# Autodesk Inventor assembly: Carriage_Assembly
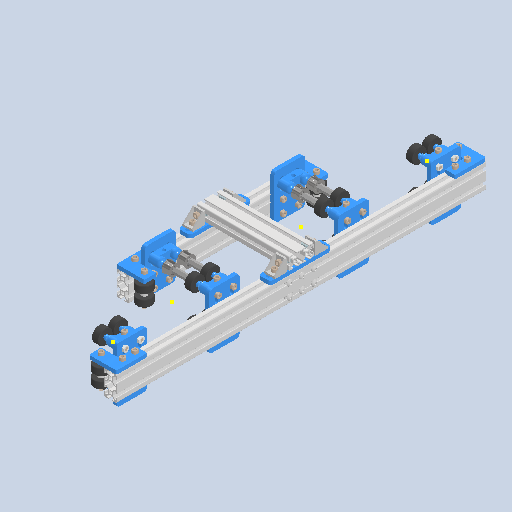
[picture p0: Inventor's stored thumbnail of the model, 512x512]
Saved by Autodesk Inventor 2022 (Build 260153000, 153)
## iProperties
Created: 2021-09-08
Part Number: Carriage_Assembly
Document SubType Name: Assembly
Designer: Jorian Brusind
Author: Jorian Brusind
## Documents named in this file (16)
- C:\Users\Jorian Brusind\Documents\GitHub\HyperRail\Inventor Files\Carriage_Assembly.iam
- C:\Users\Jorian Brusind\Documents\GitHub\HyperRail\Inventor Files\8020_Sets\IPT_20_Series\IPT_20_Series\20-2040_150mm.ipt
- C:\Users\Jorian Brusind\Documents\GitHub\HyperRail\Inventor Files\8020_Sets\IPT_20_Series\Extra_20_Series\8020_14056m\14056_m.ipt
- C:\Users\Jorian Brusind\Documents\GitHub\HyperRail\Inventor Files\Buffer.iam
- C:\Users\Jorian Brusind\Documents\GitHub\HyperRail\Inventor Files\Metric Spacer_Standoffs\hex spacer standoff nut M5 L30.ipt
- C:\Users\Jorian Brusind\Documents\GitHub\HyperRail\Inventor Files\Carriage_Horizontal_Spacer.ipt
- C:\Users\Jorian Brusind\Documents\GitHub\HyperRail\Inventor Files\8020_Sets\IPT_20_Series\IPT_20_Series\20-2040_400mm.ipt
- C:\Users\Jorian Brusind\Documents\GitHub\HyperRail\Inventor Files\Buffer_L.iam
- C:\Users\Jorian Brusind\Documents\GitHub\HyperRail\Inventor Files\Metric bolt\Bolt M5 10mm.ipt
- C:\Users\Jorian Brusind\Documents\GitHub\HyperRail\Inventor Files\din-508-t-slot-nut-t-nut-m4-m42-2.snapshot.3\STEPS\DIN 508, T-Slot Nut M5.ipt
- C:\Users\Jorian Brusind\Documents\GitHub\HyperRail\Inventor Files\8020_Sets\IPT_20_Series\IPT_20_Series\20-2040_300mm.ipt
- C:\Users\Jorian Brusind\Documents\GitHub\HyperRail\Inventor Files\5537T425_T-SLOTTED FRAMING.ipt
- C:\Users\Jorian Brusind\Documents\GitHub\HyperRail\Inventor Files\X_CarriageFWD_V2_1.iam
- C:\Users\Jorian Brusind\Documents\GitHub\HyperRail\Inventor Files\X_CarriageFWDBearing_V2_1_Short.iam
- C:\Users\Jorian Brusind\Documents\GitHub\HyperRail\Inventor Files\X_CarriageBWD_V2_0.iam
- C:\Users\Jorian Brusind\Documents\GitHub\HyperRail\Inventor Files\Metric bolt\Bolt M5 12mm.ipt
## Components (106 placed, 15 different names)
1. 20-2040_150mm:1 — Mate:20, Mate:21, Mate:22, Mate:23, Mate:80, Flush:33, Flush:94, Flush:96, Flush:99, Flush:102, Flush:114, Flush:124, Mate:311, Flush:186
2. 14056_m:1 — Mate:21, Flush:26, Flush:38, Mate:167, Mate:170, Mate:376, Mate:377
3. 14056_m:2 — Mate:20, Flush:26, Mate:70, Flush:37, Mate:164, Mate:165, Mate:379
4. 14056_m:3 — Mate:22, Flush:13, Mate:156, Mate:158, Flush:115, Mate:383
5. 14056_m:4 — Mate:23, Flush:13, Mate:72, Mate:159, Mate:161, Flush:114, Flush:115, Flush:116, Mate:381
6. Buffer:2 [sub-assembly] — Mate:86, Flush:55, Mate:202, Mate:203, Mate:206, Mate:207, Flush:120, Mate:293
7. Buffer:3 [sub-assembly] — Mate:196, Mate:197, Mate:198, Mate:199, Flush:127, Flush:128, Mate:310, Mate:368
8. Carriage_Horizontal_Spacer:1 — Mate:72, Mate:79, Mate:80, Flush:116, Flush:117
9. Carriage_Horizontal_Spacer:2 — Mate:70, Flush:37, Flush:38, Flush:117, Mate:290, Flush:123
10. 20-2040_400mm:1 — Mate:75, Mate:76, Mate:79, Flush:33, Mate:86, Flush:55, Mate:140, Flush:71, Flush:97, Flush:98, Flush:100, Flush:101, Flush:103, Flush:104, Flush:118, Flush:120, Mate:291, Mate:292, Flush:129, Flush:130, Mate:355, Mate:364, Flush:185, Flush:186
11. hex spacer standoff nut M5 L30:1 — Mate:295, Mate:305
12. hex spacer standoff nut M5 L30:2 — Mate:298, Mate:302
13. hex spacer standoff nut M5 L30:3 — Mate:296, Mate:306
14. hex spacer standoff nut M5 L30:4 — Mate:297, Mate:301
15. Buffer_L:1 [sub-assembly] — Mate:192, Mate:193, Mate:194, Mate:195, Flush:125, Flush:126, Mate:309, Mate:367
16. Buffer_L:2 [sub-assembly] — Mate:140, Flush:71, Mate:200, Mate:201, Mate:204, Mate:205, Flush:118, Mate:294
17. Bolt M5 10mm:1 — Mate:156, Mate:158, Mate:231
18. Bolt M5 10mm:3 — Mate:164, Mate:165, Mate:227
19. Bolt M5 10mm:6 — Mate:167, Mate:170, Mate:224
20. Bolt M5 10mm:8 — Mate:159, Mate:161, Mate:233
21. Bolt M5 10mm:9 — Mate:192, Mate:195, Mate:225
22. Bolt M5 10mm:10 — Mate:193, Mate:194, Mate:226
23. Bolt M5 10mm:11 — Mate:202, Mate:206, Mate:230
24. Bolt M5 10mm:12 — Mate:201, Mate:205, Mate:236
25. Bolt M5 10mm:13 — Mate:203, Mate:207, Mate:229
26. Bolt M5 10mm:14 — Mate:200, Mate:204, Mate:235
27. Bolt M5 10mm:15 — Mate:197, Mate:198, Mate:371
28. Bolt M5 10mm:16 — Mate:196, Mate:199, Mate:220
29. DIN 508, T-Slot Nut M5:1 — Mate:220, Mate:370
30. DIN 508, T-Slot Nut M5:2 — Mate:373, Mate:375
31. DIN 508, T-Slot Nut M5:4 — Mate:225
32. DIN 508, T-Slot Nut M5:5 — Mate:226, Mate:369
33. DIN 508, T-Slot Nut M5:6 — Mate:227, Flush:96
34. DIN 508, T-Slot Nut M5:7 — Mate:224, Flush:94
35. DIN 508, T-Slot Nut M5:8 — Mate:374, Mate:378
36. DIN 508, T-Slot Nut M5:10 — Mate:229, Flush:98
37. DIN 508, T-Slot Nut M5:11 — Mate:230, Flush:97
38. DIN 508, T-Slot Nut M5:12 — Flush:100, Mate:382
39. DIN 508, T-Slot Nut M5:13 — Mate:231, Flush:99
40. DIN 508, T-Slot Nut M5:14 — Mate:233, Flush:102
41. DIN 508, T-Slot Nut M5:15 — Flush:101, Mate:380
42. DIN 508, T-Slot Nut M5:16 — Mate:235, Flush:103
43. DIN 508, T-Slot Nut M5:17 — Mate:236, Flush:104
44. 20-2040_300mm:1 — Mate:283, Mate:284, Mate:285, Mate:286, Mate:287, Mate:288, Mate:289, Flush:121, Flush:122, Mate:290, Flush:123, Flush:124, Flush:127, Flush:128, Mate:299, Mate:308, Mate:311, Mate:318, Mate:319, Mate:368, Mate:370, Mate:372, Mate:373
45. 20-2040_300mm:2 — Mate:289, Flush:121, Flush:122, Flush:125, Flush:126, Mate:300, Mate:307, Mate:346, Flush:185, Mate:367, Mate:369, Mate:374, Mate:384, Mate:385
46. 5537T425_T-SLOTTED FRAMING:1 — Mate:283, Mate:284, Mate:285
47. 5537T425_T-SLOTTED FRAMING:2 — Mate:286, Mate:287, Mate:288
48. X_CarriageFWD_V2_1:1 [sub-assembly] — Mate:300, Mate:301, Mate:302, Flush:133, Mate:303, Flush:134, Flush:137, Flush:138, Flush:139, Flush:140, Mate:334, Mate:335, Mate:336, Mate:337, Mate:366, Flush:188, Flush:189, Flush:193
49. X_CarriageFWD_V2_1:2 [sub-assembly] — Mate:299, Mate:304, Mate:305, Mate:306, Flush:135, Flush:136, Flush:137, Flush:140, Flush:141, Flush:143, Mate:316, Mate:317, Mate:320, Mate:321, Flush:187, Flush:188, Flush:193
50. X_CarriageFWDBearing_V2_1_Short:1 [sub-assembly] — Mate:291, Flush:129, Mate:293, Mate:297, Mate:298, Flush:133, Mate:303, Flush:142, Mate:351, Mate:352, Mate:353, Mate:354
51. X_CarriageFWDBearing_V2_1_Short:2 [sub-assembly] — Mate:292, Flush:130, Mate:294, Mate:295, Mate:296, Mate:304, Flush:142, Flush:143, Mate:360, Mate:361, Mate:362, Mate:363, Mate:365
52. X_CarriageBWD_V2_0:1 [sub-assembly] — Mate:307, Flush:134, Mate:309, Flush:138, Flush:139, Mate:342, Mate:343, Mate:344, Mate:345, Flush:189
53. X_CarriageBWD_V2_0:2 [sub-assembly] — Mate:308, Flush:135, Mate:310, Flush:136, Flush:141, Mate:326, Mate:327, Mate:328, Mate:329, Flush:187
54. Bolt M5 10mm:17 — Mate:316, Flush:180
55. DIN 508, T-Slot Nut M5:18 — Mate:318
56. Bolt M5 10mm:18 — Mate:317, Flush:179, Flush:181
57. DIN 508, T-Slot Nut M5:19 — Mate:319
58. Bolt M5 10mm:19 — Mate:320, Flush:178
59. DIN 508, T-Slot Nut M5:20 — Flush:147, Flush:148, Flush:156
60. Bolt M5 10mm:20 — Mate:321, Flush:177, Flush:178, Flush:179, Flush:180
61. DIN 508, T-Slot Nut M5:21 — Flush:148
62. Bolt M5 10mm:21 — Mate:327, Flush:182
63. DIN 508, T-Slot Nut M5:22 — Flush:146
64. Bolt M5 10mm:22 — Mate:329, Flush:181, Flush:182, Flush:183, Flush:184
65. DIN 508, T-Slot Nut M5:23 — Flush:145, Flush:146
66. Bolt M5 10mm:23 — Mate:326, Flush:184
67. DIN 508, T-Slot Nut M5:24 — Flush:144, Flush:145
68. Bolt M5 10mm:24 — Mate:328, Flush:183
69. DIN 508, T-Slot Nut M5:25 — Flush:144, Flush:147
70. Bolt M5 10mm:25 — Mate:334, Flush:170, Mate:385
71. DIN 508, T-Slot Nut M5:26 — Flush:154, Flush:155
72. Bolt M5 10mm:26 — Mate:335, Flush:172
73. DIN 508, T-Slot Nut M5:27 — Flush:155, Flush:156
74. Bolt M5 10mm:27 — Mate:336, Mate:366, Flush:170, Flush:171, Flush:172, Flush:173, Mate:384
75. DIN 508, T-Slot Nut M5:28 — Flush:153, Flush:154
76. Bolt M5 10mm:28 — Mate:337, Flush:171, Flush:177
77. DIN 508, T-Slot Nut M5:29 — Flush:152, Flush:153
78. Bolt M5 10mm:29 — Mate:342, Flush:174
79. DIN 508, T-Slot Nut M5:30 — Flush:150, Flush:151, Flush:152
80. Bolt M5 10mm:30 — Mate:343, Flush:173, Flush:174, Flush:175, Flush:176
81. DIN 508, T-Slot Nut M5:31 — Flush:150
82. Bolt M5 10mm:31 — Mate:344, Flush:176
83. DIN 508, T-Slot Nut M5:32 — Flush:149, Flush:151
84. Bolt M5 10mm:32 — Mate:345, Flush:175
85. DIN 508, T-Slot Nut M5:33 — Flush:149, Mate:346
86. Bolt M5 10mm:33 — Mate:353, Flush:168
87. DIN 508, T-Slot Nut M5:34
88. Bolt M5 10mm:34 — Mate:351, Flush:167
89. DIN 508, T-Slot Nut M5:35
90. Bolt M5 10mm:35 — Mate:354, Flush:169
91. DIN 508, T-Slot Nut M5:36 — Mate:355
92. Bolt M5 10mm:36 — Mate:352, Flush:166, Flush:167, Flush:168, Flush:169
93. DIN 508, T-Slot Nut M5:37
94. Bolt M5 10mm:37 — Mate:360, Flush:165
95. DIN 508, T-Slot Nut M5:38
96. Bolt M5 10mm:38 — Mate:361, Mate:365, Flush:163, Flush:164, Flush:165, Flush:166
97. DIN 508, T-Slot Nut M5:39
98. Bolt M5 10mm:39 — Mate:363, Flush:164
99. DIN 508, T-Slot Nut M5:40
100. Bolt M5 10mm:40 — Mate:362, Flush:163
101. DIN 508, T-Slot Nut M5:41 — Mate:364
102. DIN 508, T-Slot Nut M5:42 — Mate:371, Mate:372
103. Bolt M5 12mm:1 — Mate:380, Mate:381, Flush:191, Flush:192
104. Bolt M5 12mm:2 — Mate:382, Mate:383, Flush:192
105. Bolt M5 12mm:3 — Mate:378, Mate:379, Flush:190
106. Bolt M5 12mm:4 — Mate:375, Mate:376, Mate:377, Flush:190, Flush:191
## Relationships (244: Mate 150, Flush 94)
- Mate:20 (3 mm): 20-2040_150mm:1 ↔ 14056_m:2
- Mate:21 (3 mm): 20-2040_150mm:1 ↔ 14056_m:1
- Mate:22 (3 mm): 20-2040_150mm:1 ↔ 14056_m:3
- Mate:23 (3 mm): 20-2040_150mm:1 ↔ 14056_m:4
- Flush:13: 14056_m:3 ↔ 14056_m:4
- Flush:26: 14056_m:1 ↔ 14056_m:2
- Mate:70: 14056_m:2 ↔ Carriage_Horizontal_Spacer:2
- Mate:72: 14056_m:4 ↔ Carriage_Horizontal_Spacer:1
- Mate:75: 20-2040_400mm:1
- Mate:76: 20-2040_400mm:1
- Mate:79: Carriage_Horizontal_Spacer:1 ↔ 20-2040_400mm:1
- Mate:80: 20-2040_150mm:1 ↔ Carriage_Horizontal_Spacer:1
- Flush:33: 20-2040_150mm:1 ↔ 20-2040_400mm:1
- Flush:37: 14056_m:2 ↔ Carriage_Horizontal_Spacer:2
- Flush:38: 14056_m:1 ↔ Carriage_Horizontal_Spacer:2
- Mate:86: Buffer:2 ↔ 20-2040_400mm:1
- Flush:55: Buffer:2 ↔ 20-2040_400mm:1
- Mate:140: 20-2040_400mm:1 ↔ Buffer_L:2
- Flush:71: 20-2040_400mm:1 ↔ Buffer_L:2
- Mate:156: 14056_m:3 ↔ Bolt M5 10mm:1
- Mate:158: 14056_m:3 ↔ Bolt M5 10mm:1
- Mate:159: 14056_m:4 ↔ Bolt M5 10mm:8
- Mate:161: 14056_m:4 ↔ Bolt M5 10mm:8
- Mate:164: 14056_m:2 ↔ Bolt M5 10mm:3
- Mate:165: 14056_m:2 ↔ Bolt M5 10mm:3
- Mate:167: 14056_m:1 ↔ Bolt M5 10mm:6
- Mate:170: 14056_m:1 ↔ Bolt M5 10mm:6
- Mate:192: Buffer_L:1 ↔ Bolt M5 10mm:9
- Mate:193: Buffer_L:1 ↔ Bolt M5 10mm:10
- Mate:194: Buffer_L:1 ↔ Bolt M5 10mm:10
- Mate:195: Buffer_L:1 ↔ Bolt M5 10mm:9
- Mate:196: Buffer:3 ↔ Bolt M5 10mm:16
- Mate:197: Buffer:3 ↔ Bolt M5 10mm:15
- Mate:198: Buffer:3 ↔ Bolt M5 10mm:15
- Mate:199: Buffer:3 ↔ Bolt M5 10mm:16
- Mate:200: Buffer_L:2 ↔ Bolt M5 10mm:14
- Mate:201: Buffer_L:2 ↔ Bolt M5 10mm:12
- Mate:202: Buffer:2 ↔ Bolt M5 10mm:11
- Mate:203: Buffer:2 ↔ Bolt M5 10mm:13
- Mate:204: Buffer_L:2 ↔ Bolt M5 10mm:14
- Mate:205: Buffer_L:2 ↔ Bolt M5 10mm:12
- Mate:206: Buffer:2 ↔ Bolt M5 10mm:11
- Mate:207: Buffer:2 ↔ Bolt M5 10mm:13
- Mate:220: Bolt M5 10mm:16 ↔ DIN 508, T-Slot Nut M5:1
- Mate:224: Bolt M5 10mm:6 ↔ DIN 508, T-Slot Nut M5:7
- Mate:225: Bolt M5 10mm:9 ↔ DIN 508, T-Slot Nut M5:4
- Mate:226: Bolt M5 10mm:10 ↔ DIN 508, T-Slot Nut M5:5
- Flush:94: 20-2040_150mm:1 ↔ DIN 508, T-Slot Nut M5:7
- Mate:227: Bolt M5 10mm:3 ↔ DIN 508, T-Slot Nut M5:6
- Flush:96: 20-2040_150mm:1 ↔ DIN 508, T-Slot Nut M5:6
- Mate:229: Bolt M5 10mm:13 ↔ DIN 508, T-Slot Nut M5:10
- Mate:230: Bolt M5 10mm:11 ↔ DIN 508, T-Slot Nut M5:11
- Flush:97: 20-2040_400mm:1 ↔ DIN 508, T-Slot Nut M5:11
- Flush:98: 20-2040_400mm:1 ↔ DIN 508, T-Slot Nut M5:10
- Mate:231: Bolt M5 10mm:1 ↔ DIN 508, T-Slot Nut M5:13
- Flush:99: 20-2040_150mm:1 ↔ DIN 508, T-Slot Nut M5:13
- Flush:100: 20-2040_400mm:1 ↔ DIN 508, T-Slot Nut M5:12
- Mate:233: Bolt M5 10mm:8 ↔ DIN 508, T-Slot Nut M5:14
- Flush:101: 20-2040_400mm:1 ↔ DIN 508, T-Slot Nut M5:15
- Flush:102: 20-2040_150mm:1 ↔ DIN 508, T-Slot Nut M5:14
- Mate:235: Bolt M5 10mm:14 ↔ DIN 508, T-Slot Nut M5:16
- Flush:103: 20-2040_400mm:1 ↔ DIN 508, T-Slot Nut M5:16
- Mate:236: Bolt M5 10mm:12 ↔ DIN 508, T-Slot Nut M5:17
- Flush:104: 20-2040_400mm:1 ↔ DIN 508, T-Slot Nut M5:17
- Flush:114: 20-2040_150mm:1 ↔ 14056_m:4
- Flush:115: 14056_m:3 ↔ 14056_m:4
- Flush:116 (-7 mm): 14056_m:4 ↔ Carriage_Horizontal_Spacer:1
- Flush:117: Carriage_Horizontal_Spacer:1 ↔ Carriage_Horizontal_Spacer:2
- Flush:118: 20-2040_400mm:1 ↔ Buffer_L:2
- Flush:120: Buffer:2 ↔ 20-2040_400mm:1
- Mate:283 (-1.5 mm): 20-2040_300mm:1 ↔ 5537T425_T-SLOTTED FRAMING:1
- Mate:284: 20-2040_300mm:1 ↔ 5537T425_T-SLOTTED FRAMING:1
- Mate:285: 20-2040_300mm:1 ↔ 5537T425_T-SLOTTED FRAMING:1
- Mate:286 (-1.5 mm): 20-2040_300mm:1 ↔ 5537T425_T-SLOTTED FRAMING:2
- Mate:287: 20-2040_300mm:1 ↔ 5537T425_T-SLOTTED FRAMING:2
- Mate:288: 20-2040_300mm:1 ↔ 5537T425_T-SLOTTED FRAMING:2
- Mate:289: 20-2040_300mm:1 ↔ 20-2040_300mm:2
- Flush:121: 20-2040_300mm:1 ↔ 20-2040_300mm:2
- Flush:122: 20-2040_300mm:1 ↔ 20-2040_300mm:2
- Mate:290: Carriage_Horizontal_Spacer:2 ↔ 20-2040_300mm:1
- Flush:123: Carriage_Horizontal_Spacer:2 ↔ 20-2040_300mm:1
- Flush:124: 20-2040_150mm:1 ↔ 20-2040_300mm:1
- Flush:125: Buffer_L:1 ↔ 20-2040_300mm:2
- Flush:126: Buffer_L:1 ↔ 20-2040_300mm:2
- Flush:127: Buffer:3 ↔ 20-2040_300mm:1
- Flush:128: Buffer:3 ↔ 20-2040_300mm:1
- Mate:291: 20-2040_400mm:1 ↔ X_CarriageFWDBearing_V2_1_Short:1
- Mate:292: 20-2040_400mm:1 ↔ X_CarriageFWDBearing_V2_1_Short:2
- Flush:129: 20-2040_400mm:1 ↔ X_CarriageFWDBearing_V2_1_Short:1
- Flush:130: 20-2040_400mm:1 ↔ X_CarriageFWDBearing_V2_1_Short:2
- Mate:293: Buffer:2 ↔ X_CarriageFWDBearing_V2_1_Short:1
- Mate:294: Buffer_L:2 ↔ X_CarriageFWDBearing_V2_1_Short:2
- Mate:295: hex spacer standoff nut M5 L30:1 ↔ X_CarriageFWDBearing_V2_1_Short:2
- Mate:296: hex spacer standoff nut M5 L30:3 ↔ X_CarriageFWDBearing_V2_1_Short:2
- Mate:297: hex spacer standoff nut M5 L30:4 ↔ X_CarriageFWDBearing_V2_1_Short:1
- Mate:298: hex spacer standoff nut M5 L30:2 ↔ X_CarriageFWDBearing_V2_1_Short:1
- Mate:299: 20-2040_300mm:1 ↔ X_CarriageFWD_V2_1:2
- Mate:300: 20-2040_300mm:2 ↔ X_CarriageFWD_V2_1:1
- Mate:301: hex spacer standoff nut M5 L30:4 ↔ X_CarriageFWD_V2_1:1
- Mate:302: hex spacer standoff nut M5 L30:2 ↔ X_CarriageFWD_V2_1:1
- Flush:133: X_CarriageFWD_V2_1:1 ↔ X_CarriageFWDBearing_V2_1_Short:1
- Mate:303: X_CarriageFWD_V2_1:1 ↔ X_CarriageFWDBearing_V2_1_Short:1
- Mate:304: X_CarriageFWD_V2_1:2 ↔ X_CarriageFWDBearing_V2_1_Short:2
- Mate:305: hex spacer standoff nut M5 L30:1 ↔ X_CarriageFWD_V2_1:2
- Mate:306: hex spacer standoff nut M5 L30:3 ↔ X_CarriageFWD_V2_1:2
- Mate:307: 20-2040_300mm:2 ↔ X_CarriageBWD_V2_0:1
- Mate:308: 20-2040_300mm:1 ↔ X_CarriageBWD_V2_0:2
- Flush:134: X_CarriageFWD_V2_1:1 ↔ X_CarriageBWD_V2_0:1
- Flush:135: X_CarriageFWD_V2_1:2 ↔ X_CarriageBWD_V2_0:2
- Mate:309: Buffer_L:1 ↔ X_CarriageBWD_V2_0:1
- Mate:310: Buffer:3 ↔ X_CarriageBWD_V2_0:2
- Flush:136: X_CarriageFWD_V2_1:2 ↔ X_CarriageBWD_V2_0:2
- Flush:137: X_CarriageFWD_V2_1:1 ↔ X_CarriageFWD_V2_1:2
- Flush:138: X_CarriageFWD_V2_1:1 ↔ X_CarriageBWD_V2_0:1
- Flush:139: X_CarriageFWD_V2_1:1 ↔ X_CarriageBWD_V2_0:1
- Flush:140: X_CarriageFWD_V2_1:1 ↔ X_CarriageFWD_V2_1:2
- Flush:141: X_CarriageFWD_V2_1:2 ↔ X_CarriageBWD_V2_0:2
- Flush:142: X_CarriageFWDBearing_V2_1_Short:1 ↔ X_CarriageFWDBearing_V2_1_Short:2
- Flush:143: X_CarriageFWD_V2_1:2 ↔ X_CarriageFWDBearing_V2_1_Short:2
- Mate:311 (-20 mm): 20-2040_150mm:1 ↔ 20-2040_300mm:1
- [Mate]: Bolt M5 10mm:17 ↔ DIN 508, T-Slot Nut M5:18
- [Mate]: Bolt M5 10mm:18 ↔ DIN 508, T-Slot Nut M5:19
- [Mate]: Bolt M5 10mm:19 ↔ DIN 508, T-Slot Nut M5:20
- [Mate]: Bolt M5 10mm:20 ↔ DIN 508, T-Slot Nut M5:21
- Mate:316: X_CarriageFWD_V2_1:2 ↔ Bolt M5 10mm:17
- Mate:317: X_CarriageFWD_V2_1:2 ↔ Bolt M5 10mm:18
- Mate:318: 20-2040_300mm:1 ↔ DIN 508, T-Slot Nut M5:18
- Mate:319: 20-2040_300mm:1 ↔ DIN 508, T-Slot Nut M5:19
- Mate:320: X_CarriageFWD_V2_1:2 ↔ Bolt M5 10mm:19
- Mate:321: X_CarriageFWD_V2_1:2 ↔ Bolt M5 10mm:20
- [Mate]: Bolt M5 10mm:21 ↔ DIN 508, T-Slot Nut M5:22
- [Mate]: Bolt M5 10mm:22 ↔ DIN 508, T-Slot Nut M5:23
- [Mate]: Bolt M5 10mm:23 ↔ DIN 508, T-Slot Nut M5:24
- [Mate]: Bolt M5 10mm:24 ↔ DIN 508, T-Slot Nut M5:25
- Mate:326: X_CarriageBWD_V2_0:2 ↔ Bolt M5 10mm:23
- Mate:327: X_CarriageBWD_V2_0:2 ↔ Bolt M5 10mm:21
- Mate:328: X_CarriageBWD_V2_0:2 ↔ Bolt M5 10mm:24
- Mate:329: X_CarriageBWD_V2_0:2 ↔ Bolt M5 10mm:22
- Flush:144: DIN 508, T-Slot Nut M5:24 ↔ DIN 508, T-Slot Nut M5:25
- Flush:145: DIN 508, T-Slot Nut M5:23 ↔ DIN 508, T-Slot Nut M5:24
- Flush:146: DIN 508, T-Slot Nut M5:22 ↔ DIN 508, T-Slot Nut M5:23
- Flush:147: DIN 508, T-Slot Nut M5:20 ↔ DIN 508, T-Slot Nut M5:25
- Flush:148: DIN 508, T-Slot Nut M5:20 ↔ DIN 508, T-Slot Nut M5:21
- [Mate]: Bolt M5 10mm:25 ↔ DIN 508, T-Slot Nut M5:26
- [Mate]: Bolt M5 10mm:26 ↔ DIN 508, T-Slot Nut M5:27
- [Mate]: Bolt M5 10mm:27 ↔ DIN 508, T-Slot Nut M5:28
- [Mate]: Bolt M5 10mm:28 ↔ DIN 508, T-Slot Nut M5:29
- Mate:334: X_CarriageFWD_V2_1:1 ↔ Bolt M5 10mm:25
- Mate:335: X_CarriageFWD_V2_1:1 ↔ Bolt M5 10mm:26
- Mate:336: X_CarriageFWD_V2_1:1 ↔ Bolt M5 10mm:27
- Mate:337: X_CarriageFWD_V2_1:1 ↔ Bolt M5 10mm:28
- [Mate]: Bolt M5 10mm:29 ↔ DIN 508, T-Slot Nut M5:30
- [Mate]: Bolt M5 10mm:30 ↔ DIN 508, T-Slot Nut M5:31
- [Mate]: Bolt M5 10mm:31 ↔ DIN 508, T-Slot Nut M5:32
- [Mate]: Bolt M5 10mm:32 ↔ DIN 508, T-Slot Nut M5:33
- Mate:342: X_CarriageBWD_V2_0:1 ↔ Bolt M5 10mm:29
- Mate:343: X_CarriageBWD_V2_0:1 ↔ Bolt M5 10mm:30
- Mate:344: X_CarriageBWD_V2_0:1 ↔ Bolt M5 10mm:31
- Mate:345: X_CarriageBWD_V2_0:1 ↔ Bolt M5 10mm:32
- Flush:149: DIN 508, T-Slot Nut M5:32 ↔ DIN 508, T-Slot Nut M5:33
- Flush:150: DIN 508, T-Slot Nut M5:30 ↔ DIN 508, T-Slot Nut M5:31
- Flush:151: DIN 508, T-Slot Nut M5:30 ↔ DIN 508, T-Slot Nut M5:32
- Flush:152: DIN 508, T-Slot Nut M5:29 ↔ DIN 508, T-Slot Nut M5:30
- Flush:153: DIN 508, T-Slot Nut M5:28 ↔ DIN 508, T-Slot Nut M5:29
- Flush:154: DIN 508, T-Slot Nut M5:26 ↔ DIN 508, T-Slot Nut M5:28
- Flush:155: DIN 508, T-Slot Nut M5:26 ↔ DIN 508, T-Slot Nut M5:27
- Flush:156: DIN 508, T-Slot Nut M5:20 ↔ DIN 508, T-Slot Nut M5:27
- Mate:346: 20-2040_300mm:2 ↔ DIN 508, T-Slot Nut M5:33
- [Mate]: Bolt M5 10mm:33 ↔ DIN 508, T-Slot Nut M5:34
- [Mate]: Bolt M5 10mm:34 ↔ DIN 508, T-Slot Nut M5:35
- [Mate]: Bolt M5 10mm:35 ↔ DIN 508, T-Slot Nut M5:36
- [Mate]: Bolt M5 10mm:36 ↔ DIN 508, T-Slot Nut M5:37
- [Flush]: DIN 508, T-Slot Nut M5:36 ↔ DIN 508, T-Slot Nut M5:37
- [Flush]: DIN 508, T-Slot Nut M5:34 ↔ DIN 508, T-Slot Nut M5:36
- [Flush]: DIN 508, T-Slot Nut M5:34 ↔ DIN 508, T-Slot Nut M5:35
- Mate:351: X_CarriageFWDBearing_V2_1_Short:1 ↔ Bolt M5 10mm:34
- Mate:352: X_CarriageFWDBearing_V2_1_Short:1 ↔ Bolt M5 10mm:36
- Mate:353: X_CarriageFWDBearing_V2_1_Short:1 ↔ Bolt M5 10mm:33
- Mate:354: X_CarriageFWDBearing_V2_1_Short:1 ↔ Bolt M5 10mm:35
- Mate:355: 20-2040_400mm:1 ↔ DIN 508, T-Slot Nut M5:36
- [Mate]: Bolt M5 10mm:37 ↔ DIN 508, T-Slot Nut M5:38
- [Mate]: Bolt M5 10mm:38 ↔ DIN 508, T-Slot Nut M5:39
- [Mate]: Bolt M5 10mm:39 ↔ DIN 508, T-Slot Nut M5:40
- [Mate]: Bolt M5 10mm:40 ↔ DIN 508, T-Slot Nut M5:41
- [Flush]: DIN 508, T-Slot Nut M5:40 ↔ DIN 508, T-Slot Nut M5:41
- [Flush]: DIN 508, T-Slot Nut M5:38 ↔ DIN 508, T-Slot Nut M5:40
- [Flush]: DIN 508, T-Slot Nut M5:38 ↔ DIN 508, T-Slot Nut M5:39
- Mate:360: X_CarriageFWDBearing_V2_1_Short:2 ↔ Bolt M5 10mm:37
- Mate:361: X_CarriageFWDBearing_V2_1_Short:2 ↔ Bolt M5 10mm:38
- Mate:362: X_CarriageFWDBearing_V2_1_Short:2 ↔ Bolt M5 10mm:40
- Mate:363: X_CarriageFWDBearing_V2_1_Short:2 ↔ Bolt M5 10mm:39
- Mate:364: 20-2040_400mm:1 ↔ DIN 508, T-Slot Nut M5:41
- Mate:365: X_CarriageFWDBearing_V2_1_Short:2 ↔ Bolt M5 10mm:38
- Flush:163: Bolt M5 10mm:38 ↔ Bolt M5 10mm:40
- Flush:164: Bolt M5 10mm:38 ↔ Bolt M5 10mm:39
- Flush:165: Bolt M5 10mm:37 ↔ Bolt M5 10mm:38
- Flush:166: Bolt M5 10mm:36 ↔ Bolt M5 10mm:38
- Flush:167: Bolt M5 10mm:34 ↔ Bolt M5 10mm:36
- Flush:168: Bolt M5 10mm:33 ↔ Bolt M5 10mm:36
- Flush:169: Bolt M5 10mm:35 ↔ Bolt M5 10mm:36
- Mate:366: X_CarriageFWD_V2_1:1 ↔ Bolt M5 10mm:27
- Flush:170: Bolt M5 10mm:25 ↔ Bolt M5 10mm:27
- Flush:171: Bolt M5 10mm:27 ↔ Bolt M5 10mm:28
- Flush:172: Bolt M5 10mm:26 ↔ Bolt M5 10mm:27
- Flush:173: Bolt M5 10mm:27 ↔ Bolt M5 10mm:30
- Flush:174: Bolt M5 10mm:29 ↔ Bolt M5 10mm:30
- Flush:175: Bolt M5 10mm:30 ↔ Bolt M5 10mm:32
- Flush:176: Bolt M5 10mm:30 ↔ Bolt M5 10mm:31
- Flush:177: Bolt M5 10mm:20 ↔ Bolt M5 10mm:28
- Flush:178: Bolt M5 10mm:19 ↔ Bolt M5 10mm:20
- Flush:179: Bolt M5 10mm:18 ↔ Bolt M5 10mm:20
- Flush:180: Bolt M5 10mm:17 ↔ Bolt M5 10mm:20
- Flush:181: Bolt M5 10mm:18 ↔ Bolt M5 10mm:22
- Flush:182: Bolt M5 10mm:21 ↔ Bolt M5 10mm:22
- Flush:183: Bolt M5 10mm:22 ↔ Bolt M5 10mm:24
- Flush:184: Bolt M5 10mm:22 ↔ Bolt M5 10mm:23
- Flush:185: 20-2040_400mm:1 ↔ 20-2040_300mm:2
- Flush:186 (130 mm): 20-2040_150mm:1 ↔ 20-2040_400mm:1
- Flush:187: X_CarriageFWD_V2_1:2 ↔ X_CarriageBWD_V2_0:2
- Flush:188: X_CarriageFWD_V2_1:1 ↔ X_CarriageFWD_V2_1:2
- Flush:189: X_CarriageFWD_V2_1:1 ↔ X_CarriageBWD_V2_0:1
- Mate:367: Buffer_L:1 ↔ 20-2040_300mm:2
- Mate:368: Buffer:3 ↔ 20-2040_300mm:1
- Mate:369: DIN 508, T-Slot Nut M5:5 ↔ 20-2040_300mm:2
- Mate:370: DIN 508, T-Slot Nut M5:1 ↔ 20-2040_300mm:1
- Mate:371: Bolt M5 10mm:15 ↔ DIN 508, T-Slot Nut M5:42
- Mate:372: 20-2040_300mm:1 ↔ DIN 508, T-Slot Nut M5:42
- Mate:373: DIN 508, T-Slot Nut M5:2 ↔ 20-2040_300mm:1
- Mate:374: DIN 508, T-Slot Nut M5:8 ↔ 20-2040_300mm:2
- Mate:375: DIN 508, T-Slot Nut M5:2 ↔ Bolt M5 12mm:4
- Mate:376: 14056_m:1 ↔ Bolt M5 12mm:4
- Mate:377: 14056_m:1 ↔ Bolt M5 12mm:4
- Mate:378: DIN 508, T-Slot Nut M5:8 ↔ Bolt M5 12mm:3
- Mate:379: 14056_m:2 ↔ Bolt M5 12mm:3
- Flush:190: Bolt M5 12mm:3 ↔ Bolt M5 12mm:4
- Mate:380: DIN 508, T-Slot Nut M5:15 ↔ Bolt M5 12mm:1
- Mate:381: 14056_m:4 ↔ Bolt M5 12mm:1
- Flush:191: Bolt M5 12mm:1 ↔ Bolt M5 12mm:4
- Mate:382: DIN 508, T-Slot Nut M5:12 ↔ Bolt M5 12mm:2
- Mate:383: 14056_m:3 ↔ Bolt M5 12mm:2
- Flush:192: Bolt M5 12mm:1 ↔ Bolt M5 12mm:2
- Mate:384 (4.25 mm): 20-2040_300mm:2 ↔ Bolt M5 10mm:27
- Mate:385 (4.25 mm): 20-2040_300mm:2 ↔ Bolt M5 10mm:25
- Flush:193: X_CarriageFWD_V2_1:1 ↔ X_CarriageFWD_V2_1:2
## Named parameters: d469_d326 = 0 mm, d470_d326 = 0 mm, d471_d326 = 0 mm, d472_d326 = 0 mm, d479_d326 = 0 mm, d480_d326 = 0 mm, d481_d326 = 0 mm, d482_d326 = 0 mm, d492_d326 = 0 mm, d493_d326 = 0 mm, d494_d326 = 0 mm, d495_d326 = 0 mm, d500_d326 = 0 mm, d501_d326 = 0 mm, d502_d326 = 0 mm, d503_d326 = 0 mm, d517_d492_d326 = 0 mm, d518_d493_d326 = 0 mm, d519_d494_d326 = 0 mm, d520_d495_d326 = 0 mm, d521_d512 = 0 mm, d522_d513 = 0 mm, d523_d514 = 0 mm, d529_d492_d326 = 0 mm, d530_d493_d326 = 0 mm, d531_d494_d326 = 0 mm, d532_d495_d326 = 0 mm, d533_d512 = 0 mm, d534_d513 = 0 mm, d535_d514 = 0 mm
